# Autodesk Inventor assembly: ProngsWithCapBall
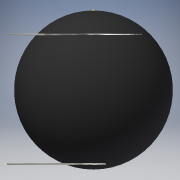
[picture p0: Inventor's stored thumbnail of the model, 180x180]
Saved by Autodesk Inventor 2017 (Build 210142000, 142)
## iProperties
Created: 2017-06-24
Part Number: ProngsWithCapBall
Document SubType Name: Assembly
Designer: User
Author: User
## Documents named in this file (4)
- C:\Robotics\CAD\2016-17_CAD\ProngsWithCapBall.iam
- C:\Robotics\CAD\2016-17_CAD\NewLiftCapBallHolderWCapBall.iam
- C:\Robotics\CAD\2016-17_CAD\PossibleTopCapBallHolder.ipt
- C:\Robotics\CAD\2016-17_CAD\LiftBallHolder.ipt
## Components (3 placed, 3 different names)
1. NewLiftCapBallHolderWCapBall:1 [sub-assembly]
2. PossibleTopCapBallHolder:1 — Flush:1
3. LiftBallHolder:1 — Flush:1
## Relationships (1: Flush 1)
- Flush:1: PossibleTopCapBallHolder:1 ↔ LiftBallHolder:1
